# Autodesk Inventor assembly: Tensioner41
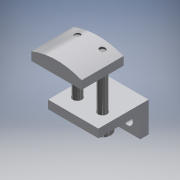
[picture p0: Inventor's stored thumbnail of the model, 180x180]
Saved by Autodesk Inventor 2017 (Build 210142000, 142)
## iProperties
Created: 2018-05-19
Part Number: Tensioner41
Document SubType Name: Assembly
Designer: User
Mass: 7.17493 g
Surface Area: 30.5775 cm^2
Volume: 3.34623 cm^3
Density: 2.14418 g/cm^3
Author: User
## Documents named in this file (4)
- C:\Robotics\CAD\2018-19_CAD\Offseason\Tensioner4a.iam
- C:\Robotics\CAD\2018-19_CAD\Offseason\TensionerPlate4a.ipt
- C:\Robotics\CAD\2018-19_CAD\Offseason\TensionerPusher4.ipt
- C:\Robotics\CAD\COTSParts\Fasteners\92012A506_.125D.75L_ALLOY STEEL PRECISION SHOULDER SCREW.ipt
## Components (4 placed, 3 different names)
1. TensionerPlate4a:1 — Mate:1, Mate:2, Mate:3
2. TensionerPusher4:1 — Insert:1, Insert:2, Mate:3
3. 92012A506_.125D.75L_ALLOY STEEL PRECISION SHOULDER SCREW:1 — Insert:2, Mate:2
4. 92012A506_.125D.75L_ALLOY STEEL PRECISION SHOULDER SCREW:2 — Insert:1, Mate:1
## Relationships (5: Mate 3, Insert 2)
- Insert:1: TensionerPusher4:1 ↔ 92012A506_.125D.75L_ALLOY STEEL PRECISION SHOULDER SCREW:2
- Insert:2: TensionerPusher4:1 ↔ 92012A506_.125D.75L_ALLOY STEEL PRECISION SHOULDER SCREW:1
- Mate:1: TensionerPlate4a:1 ↔ 92012A506_.125D.75L_ALLOY STEEL PRECISION SHOULDER SCREW:2
- Mate:2: TensionerPlate4a:1 ↔ 92012A506_.125D.75L_ALLOY STEEL PRECISION SHOULDER SCREW:1
- Mate:3: TensionerPlate4a:1 ↔ TensionerPusher4:1
